# Autodesk Inventor assembly: A_ASSEMBLY
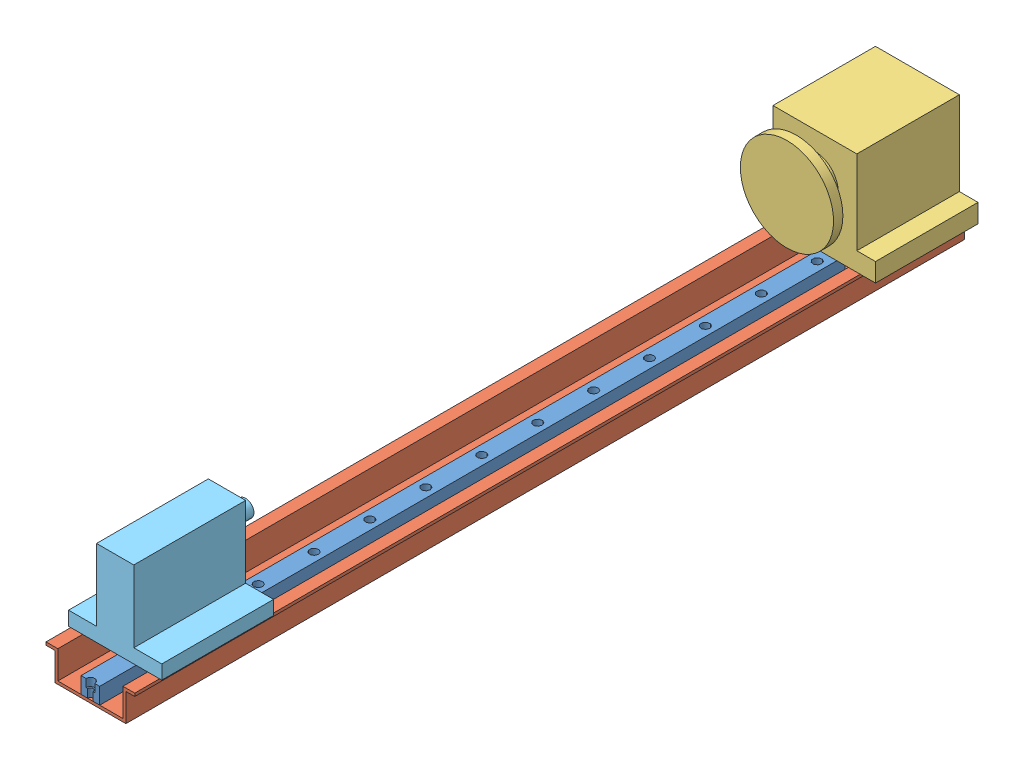
[picture p0: shaded view drawn from the shape stored in the file]
Saved by Autodesk Inventor 2023 (Build 270158000, 158)
## iProperties
Created: 2024-08-24
Part Number: A_ASSEMBLY
Document SubType Name: Assembly
Designer: think
Author: think
## Documents named in this file (6)
- G:\CNC PROJECT\CNC_Project\A_ASSEMBLY.iam
- G:\CNC PROJECT\CNC_Project\HGW20CC_Rail_800mm_ACTUAL.ipt
- G:\CNC PROJECT\CNC_Project\C_CHANNEL.ipt
- G:\CNC PROJECT\CNC_Project\HGW20CC_Slider.ipt
- G:\CNC PROJECT\CNC_Project\Tailstock.ipt
- G:\CNC PROJECT\CNC_Project\A_Gearbox.ipt
## Components (5 placed, 5 different names)
1. C_CHANNEL:1 — Mate:1, Mate:2, Flush:1, Mate:6
2. HGW20CC_Rail_800mm_ACTUAL:1 — Mate:1, Mate:2, Flush:1, Mate:3, Mate:4
3. HGW20CC_Slider:1 — Mate:3, Mate:4, Mate:5, Flush:2, Flush:3
4. Tailstock:1 — Mate:5, Flush:2, Flush:3
5. A_Gearbox:1 — Mate:6
## Relationships (9: Mate 6, Flush 3)
- Mate:1: C_CHANNEL:1 ↔ HGW20CC_Rail_800mm_ACTUAL:1
- Mate:2 (24.925 mm): C_CHANNEL:1 ↔ HGW20CC_Rail_800mm_ACTUAL:1
- Flush:1: C_CHANNEL:1 ↔ HGW20CC_Rail_800mm_ACTUAL:1
- Mate:3: HGW20CC_Rail_800mm_ACTUAL:1 ↔ HGW20CC_Slider:1
- Mate:4: HGW20CC_Rail_800mm_ACTUAL:1 ↔ HGW20CC_Slider:1
- Mate:5: HGW20CC_Slider:1 ↔ Tailstock:1
- Flush:2: HGW20CC_Slider:1 ↔ Tailstock:1
- Flush:3 (11.5 mm): HGW20CC_Slider:1 ↔ Tailstock:1
- Mate:6: C_CHANNEL:1 ↔ A_Gearbox:1
